# Autodesk Inventor assembly: Mechanical Ring
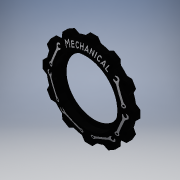
[picture p0: Inventor's stored thumbnail of the model, 180x180]
Saved by Autodesk Inventor 2016 (Build 200138000, 138)
## iProperties
Created: 2015-06-02
Part Number: Mechanical Ring
Document SubType Name: Assembly
Designer: Spooner
Author: Spooner
## Documents named in this file (5)
- C:\Users\Spooner\Documents\Inventor\2016 RoboCat\Mechanical Ring.iam
- C:\Users\Spooner\Documents\Inventor\2016 RoboCat\Team Pin Mechanical.ipt
- C:\Users\Spooner\Documents\Inventor\2016 RoboCat\Team Pin Mechanical-Text.ipt
- C:\Users\Spooner\Documents\Inventor\2016 RoboCat\Team Pin Mechanical-Left Wrench.ipt
- C:\Users\Spooner\Documents\Inventor\2016 RoboCat\Team Pin Mechanical-Right Wrench.ipt
## Components (8 placed, 4 different names)
1. Team Pin Mechanical:1 — Mate:10, Mate:11, Mate:12, Insert:3, Mate:13, Insert:4, Mate:14, Insert:5, Mate:15, Insert:6, Mate:16, Insert:7, Mate:17, Insert:8, Mate:18
2. Team Pin Mechanical-Text:1 — Mate:10, Mate:11, Mate:12
3. Team Pin Mechanical-Left Wrench:1 — Insert:4, Mate:14
4. Team Pin Mechanical-Left Wrench:2 — Insert:5, Mate:15
5. Team Pin Mechanical-Left Wrench:3 — Insert:3, Mate:13
6. Team Pin Mechanical-Right Wrench:1 — Insert:6, Mate:16
7. Team Pin Mechanical-Right Wrench:2 — Insert:7, Mate:17
8. Team Pin Mechanical-Right Wrench:3 — Insert:8, Mate:18
## Relationships (15: Mate 9, Insert 6)
- Mate:10: Team Pin Mechanical:1 ↔ Team Pin Mechanical-Text:1
- Mate:11: Team Pin Mechanical:1 ↔ Team Pin Mechanical-Text:1
- Mate:12: Team Pin Mechanical:1 ↔ Team Pin Mechanical-Text:1
- Insert:3: Team Pin Mechanical:1 ↔ Team Pin Mechanical-Left Wrench:3
- Mate:13: Team Pin Mechanical:1 ↔ Team Pin Mechanical-Left Wrench:3
- Insert:4: Team Pin Mechanical:1 ↔ Team Pin Mechanical-Left Wrench:1
- Mate:14: Team Pin Mechanical:1 ↔ Team Pin Mechanical-Left Wrench:1
- Insert:5: Team Pin Mechanical:1 ↔ Team Pin Mechanical-Left Wrench:2
- Mate:15: Team Pin Mechanical:1 ↔ Team Pin Mechanical-Left Wrench:2
- Insert:6: Team Pin Mechanical:1 ↔ Team Pin Mechanical-Right Wrench:1
- Mate:16: Team Pin Mechanical:1 ↔ Team Pin Mechanical-Right Wrench:1
- Insert:7: Team Pin Mechanical:1 ↔ Team Pin Mechanical-Right Wrench:2
- Mate:17: Team Pin Mechanical:1 ↔ Team Pin Mechanical-Right Wrench:2
- Insert:8: Team Pin Mechanical:1 ↔ Team Pin Mechanical-Right Wrench:3
- Mate:18: Team Pin Mechanical:1 ↔ Team Pin Mechanical-Right Wrench:3
